# Autodesk Inventor assembly: PDRHN50
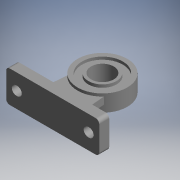
[picture p0: Inventor's stored thumbnail of the model, 180x180]
Saved by Autodesk Inventor 2017.3 (Build 213256000, 256)
## iProperties
Category: PARTsolutions
Company: MISUMI
Part Number: PDRHN50
Catalog Web Link: www.cadenas.de
Description: PDRH,PDRHN-Ball Bearing Units -High-Centered Pillow Type-
Vendor: MISUMI
Document SubType Name: Assembly
Designer: partserver
Manufacturer: MISUMI
Mass: 621.544 g
Surface Area: 938.833 cm^2
Volume: 621.544 cm^3
Density: 1 g/cm^3
Title: PDRHN50
Author: Cadenas PARTsolutions
Comments: Ball Bearing Units -High-Centered Pillow Type-
PSOL_IDENT_0: {$CADENAS_DATA\23d-libs\misumi\metric\12_bearing_holders\pdrh_asmtab.prj},175 {VTYP=3D},{STYP=ASSTAB
PSOL_IDENT_1: },{NB=PDRHN50},{LINA=PDRHN50},{NN=PDRH,PDRHN},{DATE=11.12.2019 10:07:02},{GEOMDATE=02.12.2019 09:15:
PSOL_IDENT_2: 31},{VERSION=},{LINEID=100},{WBVAR=TS},{WBNUMERIC=}  {NB=PDRHN50},{LINA=PDRHN50},{KT=DUMMY},{PN=PDRH
PSOL_IDENT_3: N50},{TYPE=PDRHN},{MATH=Cast Iron Class No.30},{MATB=52100 Bearing Steel},{MATRS=Nitrile Rubber},{MA
PSOL_IDENT_4: TSS=4137 Alloy Steel},{PRECISION=JIS B 1558/JIS B 1514/JIS B 1559},{OT=-15 ~+100},{TS=2},{TSALG='1','
PSOL_IDENT_5: Lubrication Type' , '2','Oil-Free Type'},{D=50},{JIS=UC210D1},{H=110},{L=206},{L1=159},{A=70},{DD1=2
PSOL_IDENT_6: 2},{DD=20},{TT=22},{H1=165},{B=51.6},{S=19.0},{CR=35.0},{COR=23.20},{M1=M8x1.0},{MD=8},{MPITCH=1.00}
PSOL_IDENT_7: ,{ML=10},{MASS=3900},{RLD1=110},{RLD2=90},{RLD3=62.4},{LD1=37},{LD2=6.0},{LD3=3},{G1=40.5},{G2=15.5}
PSOL_IDENT_8: ,{G3=55},{R1=16},{R2=8},{NCL=1.5},{KCL=23.6},{PPATH=pdrh/pdrh_asmtpl.prj}
NB: PDRHN50
NN: PDRH,PDRHN
NT: Ball Bearing Units -High-Centered Pillow Type-
NBSYN: $PN.
LINA: PDRHN50
CATALOG: Misumi
PN: PDRHN50
TYPE: PDRHN
MATH: Cast Iron Class No.30
MATB: 52100 Bearing Steel
MATRS: Nitrile Rubber
MATSS: 4137 Alloy Steel
PRECISION: JIS B 1558/JIS B 1514/JIS B 1559
OT: -15 ~+100
TS: Oil-Free Type
D: 50
JIS: UC210D1
H: 110
L: 206
L1: 159
A: 70
DD1: 22
DD: 20
TT: 22
H1: 165
B: 51.6
S: 19
CR: 35
COR: 23.2
M1: M8x1.0
MASS: 3900
PPATH: pdrh/pdrh_asmtpl.prj
SUPPLIER: MISUMI
ARTICLENO: PDRHN50
BOMINFO: PDRHN50
CREATOR: CADENAS GmbH
## Documents named in this file (3)
- e:\temp\worker_13\temp\exporttempdir_6896_336_NZXiV\format_0\PDRHN50.iam
- e:\temp\worker_13\temp\exporttempdir_6896_336_NZXiV\format_0\PDRHN50_b.ipt
- e:\temp\worker_13\temp\exporttempdir_6896_336_NZXiV\format_0\SET-SCREW8-10.ipt
## Components (3 placed, 2 different names)
1. PDRHN50_b:1 — CP1_XY@1 <-> CP_XY@2, CP1_Z@1 <-> CP_Z@2, CP1_YZ@1 <-> CP_YZ@2, CP2_XY@1 <-> CP_XY@3, CP2_Z@1 <-> CP_Z@3, CP2_YZ@1 <-> CP_YZ@3
2. SET-SCREW8-10:1 — CP1_XY@1 <-> CP_XY@2, CP1_Z@1 <-> CP_Z@2, CP1_YZ@1 <-> CP_YZ@2
3. SET-SCREW8-10:2 — CP2_XY@1 <-> CP_XY@3, CP2_Z@1 <-> CP_Z@3, CP2_YZ@1 <-> CP_YZ@3
## Relationships (6: Mate 4, Angle 2)
- CP1_XY@1 <-> CP_XY@2 [Mate]: PDRHN50_b:1 ↔ SET-SCREW8-10:1
- CP1_Z@1 <-> CP_Z@2 [Mate]: PDRHN50_b:1 ↔ SET-SCREW8-10:1
- CP1_YZ@1 <-> CP_YZ@2 [Angle] (0 deg): PDRHN50_b:1 ↔ SET-SCREW8-10:1
- CP2_XY@1 <-> CP_XY@3 [Mate]: PDRHN50_b:1 ↔ SET-SCREW8-10:2
- CP2_Z@1 <-> CP_Z@3 [Mate]: PDRHN50_b:1 ↔ SET-SCREW8-10:2
- CP2_YZ@1 <-> CP_YZ@3 [Angle] (0 deg): PDRHN50_b:1 ↔ SET-SCREW8-10:2
